# Autodesk Inventor assembly: Assembly
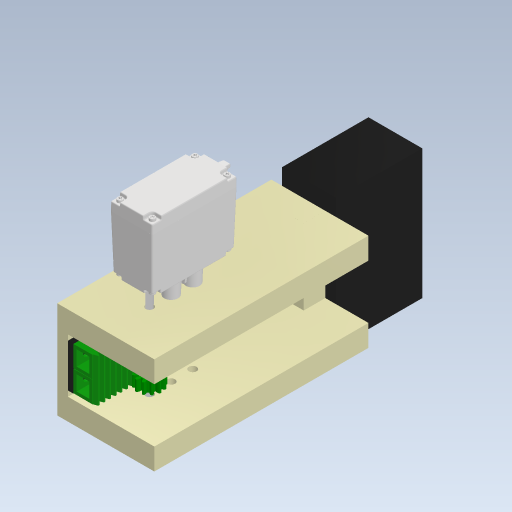
[picture p0: Inventor's stored thumbnail of the model, 512x512]
Saved by Autodesk Inventor 2024 (Build 280153000, 153)
## iProperties
Created: 2024-11-10
Part Number: Assembly
Document SubType Name: Assembly
Designer: Oscar
Author: Oscar
## Documents named in this file (7)
- C:\Users\Takum\OneDrive\Documents\GitHub\1622-2024-Assignments\Oscar - Example\EDD STUFSS\Assembly.iam
- C:\Users\Takum\OneDrive\Documents\GitHub\1622-2024-Assignments\Oscar - Example\EDD STUFSS\blocker.ipt
- C:\Users\Takum\OneDrive\Documents\GitHub\1622-2024-Assignments\Oscar - Example\EDD STUFSS\Rack Gear v2 (276-4782).ipt
- C:\Users\Takum\OneDrive\Documents\GitHub\1622-2024-Assignments\Oscar - Example\EDD STUFSS\2-Wire Motor 393 (276-2177)\2-Wire Motor 393 (276-2177).iam
- C:\Users\Takum\OneDrive\Documents\GitHub\1622-2024-Assignments\Oscar - Example\EDD STUFSS\case.ipt
- C:\Users\Takum\OneDrive\Documents\GitHub\1622-2024-Assignments\Oscar - Example\EDD STUFSS\12T Gear (276-2169-001).ipt
- C:\Users\Takum\OneDrive\Documents\GitHub\1622-2024-Assignments\Oscar - Example\EDD STUFSS\shaft.ipt
## Components (11 placed, 6 different names)
1. blocker:1 — Mate:1, Mate:2, Mate:3, Mate:4, Mate:5, Mate:6, Mate:7, Mate:8, Mate:9, Mate:10, Mate:11, Mate:12, Mate:14, Mate:24
2. Rack Gear v2 (276-4782):1 — Mate:1, Mate:2, Mate:3
3. Rack Gear v2 (276-4782):2 — Mate:4, Mate:5, Mate:11
4. Rack Gear v2 (276-4782):3 — Mate:8, Mate:9, Mate:10
5. Rack Gear v2 (276-4782):4 — Mate:6, Mate:7, Mate:12, Mate:15
6. 2-Wire Motor 393 (276-2177):1 [sub-assembly] — Mate:16, Mate:17, Mate:18, Mate:21
7. case:1 — Mate:14, Mate:15, Mate:16, Mate:17, Mate:18, Mate:19, Mate:20, Mate:24
8. 12T Gear (276-2169-001):1 — Mate:19, Mate:22
9. shaft:1 — Mate:20, Mate:21
10. 12T Gear (276-2169-001):2 — Mate:22, Mate:23
11. 12T Gear (276-2169-001):3 — Mate:23
## Relationships (23: Mate 23)
- Mate:1: blocker:1 ↔ Rack Gear v2 (276-4782):1
- Mate:2: blocker:1 ↔ Rack Gear v2 (276-4782):1
- Mate:3: blocker:1 ↔ Rack Gear v2 (276-4782):1
- Mate:4: blocker:1 ↔ Rack Gear v2 (276-4782):2
- Mate:5: blocker:1 ↔ Rack Gear v2 (276-4782):2
- Mate:6: blocker:1 ↔ Rack Gear v2 (276-4782):4
- Mate:7: blocker:1 ↔ Rack Gear v2 (276-4782):4
- Mate:8: blocker:1 ↔ Rack Gear v2 (276-4782):3
- Mate:9: blocker:1 ↔ Rack Gear v2 (276-4782):3
- Mate:10: blocker:1 ↔ Rack Gear v2 (276-4782):3
- Mate:11: blocker:1 ↔ Rack Gear v2 (276-4782):2
- Mate:12: blocker:1 ↔ Rack Gear v2 (276-4782):4
- Mate:14: blocker:1 ↔ case:1
- Mate:15 (3.175 mm): Rack Gear v2 (276-4782):4 ↔ case:1
- Mate:16: 2-Wire Motor 393 (276-2177):1 ↔ case:1
- Mate:17: 2-Wire Motor 393 (276-2177):1 ↔ case:1
- Mate:18: 2-Wire Motor 393 (276-2177):1 ↔ case:1
- Mate:19: case:1 ↔ 12T Gear (276-2169-001):1
- Mate:20: case:1 ↔ shaft:1
- Mate:21: 2-Wire Motor 393 (276-2177):1 ↔ shaft:1
- Mate:22: 12T Gear (276-2169-001):1 ↔ 12T Gear (276-2169-001):2
- Mate:23: 12T Gear (276-2169-001):2 ↔ 12T Gear (276-2169-001):3
- Mate:24: blocker:1 ↔ case:1
